# Autodesk Inventor assembly: Front_Upper_Arm_Assembly
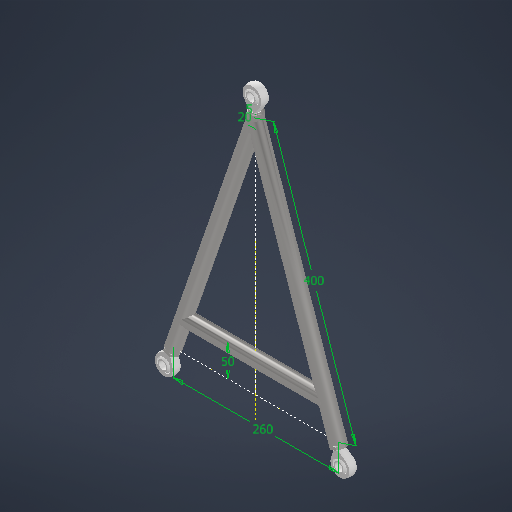
[picture p0: Inventor's stored thumbnail of the model, 512x512]
Saved by Autodesk Inventor 2026.1 (Build 301233000, 233)
## iProperties
_SolveAssemblyDoc: Frame Generator Solve Assembly
_Version: 15.0.0
Created: 2026-06-12
Part Number: Front_Upper_Arm_Assembly
Document SubType Name: Assembly
Designer: share
Author: share
## iProperties of the stored document MemberDocs/xMjmzjztqKsfgw2maZjoj4ywb1d
_SolveAssemblyDoc: Frame Generator Solve Assembly
_Version: 15.0.0
Created: 2026-06-12
Part Number: Front_Upper_Arm_Assembly
Document SubType Name: Assembly
Designer: share
Author: share
## iProperties of the stored document MemberDocs/xA44zzlwwFcqn4ttdDgc3dhpt2f
_SolveAssemblyDoc: Frame Generator Solve Assembly
_Version: 15.0.0
Created: 2026-06-12
Part Number: Front_Upper_Arm_Assembly
Document SubType Name: Assembly
Designer: share
Author: share
## iProperties of the stored document MemberDocs/xO5ksdanqL0dmwrtuTkp30e5fSb
_SolveAssemblyDoc: Frame Generator Solve Assembly
_Version: 15.0.0
Created: 2026-06-12
Part Number: Front_Upper_Arm_Assembly
Document SubType Name: Assembly
Designer: share
Author: share
## Documents named in this file (5)
- C:\Users\share\OneDrive\Documents\Personal Projects\GOGO Kart\CAD\GOGO_KART_FSAE\Suspension\Suspension Parts\Front Upper Arm\Front_Upper_Arm_Assembly.iam
- C:\Users\share\OneDrive\Documents\Personal Projects\GOGO Kart\CAD\GOGO_KART_FSAE\Suspension\Suspension Parts\Front Upper Arm\Front_Upper_Arm_Outline_Sketch.ipt
- C:\Users\share\OneDrive\Documents\Personal Projects\GOGO Kart\CAD\GOGO_KART_FSAE\Suspension\Suspension Parts\Front Upper Arm\Front_Upper_Arm_Assembly\Frame\Frame 1781239343037.iam
- C:\Users\share\OneDrive\Documents\Inventor\Content Center Files\R2026\en-US\DIN 439-2\DIN 439 - M12 x 1.25.ipt
- C:\Users\share\OneDrive\Documents\Personal Projects\GOGO Kart\CAD\GOGO_KART_FSAE\Suspension\Suspension Parts\Front Upper Arm\Rod End CAD Files\185237224-9-20263829\20263829.iam
## Components (8 placed, 4 different names)
1. Front_Upper_Arm_Outline_Sketch:1
2. Frame 1781239343037:1 [sub-assembly] — Insert:1, Insert:2, Insert:3
3. DIN 439-2 - replaced by DIN EN 24035/28675 M12 x 1.25:1 — Insert:1, Insert:6
4. DIN 439-2 - replaced by DIN EN 24035/28675 M12 x 1.25:2 — Insert:2, Insert:5
5. DIN 439-2 - replaced by DIN EN 24035/28675 M12 x 1.25:3 — Insert:3, Insert:4
6. 20263829:1 [sub-assembly] — Insert:4
7. 20263829:2 [sub-assembly] — Insert:5
8. 20263829:3 [sub-assembly] — Insert:6
## Relationships (6: Insert 6)
- Insert:1: Frame 1781239343037:1 ↔ DIN 439-2 - replaced by DIN EN 24035/28675 M12 x 1.25:1
- Insert:2: Frame 1781239343037:1 ↔ DIN 439-2 - replaced by DIN EN 24035/28675 M12 x 1.25:2
- Insert:3: Frame 1781239343037:1 ↔ DIN 439-2 - replaced by DIN EN 24035/28675 M12 x 1.25:3
- Insert:4: DIN 439-2 - replaced by DIN EN 24035/28675 M12 x 1.25:3 ↔ 20263829:1
- Insert:5: DIN 439-2 - replaced by DIN EN 24035/28675 M12 x 1.25:2 ↔ 20263829:2
- Insert:6: DIN 439-2 - replaced by DIN EN 24035/28675 M12 x 1.25:1 ↔ 20263829:3
